# Autodesk Inventor assembly: 組合3-15
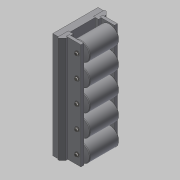
[picture p0: Inventor's stored thumbnail of the model, 180x180]
Saved by Autodesk Inventor 2018 (Build 220112000, 112)
## iProperties
Created: 2020-09-23
Part Number: 組合3-15
Material: 一般
Document SubType Name: Assembly
Designer: 王鼎鈞
Author: 王鼎鈞
## Documents named in this file (7)
- D:\2020嚴家明 功課黨\組合3-15.iam
- D:\2020嚴家明 功課黨\exercise3-11.ipt
- D:\2020嚴家明 功課黨\exercise3-12.ipt
- D:\2020嚴家明 功課黨\exercise3-13.ipt
- D:\2020嚴家明 功課黨\exercise3-14ipt.ipt
- C:\Users\王鼎鈞\Documents\Inventor\Content Center Files\R2018\zh-TW\CNS 4411\CNS 4411 - M 10 x 40.ipt
- D:\2020嚴家明 功課黨\AS 1427 - M10 x 50(4).ipt
## Components (30 placed, 6 different names)
1. exercise3-11:1 — 插入:2, 貼合:14, 插入:17, 插入:22
2. exercise3-12:1 — 貼合:9, 貼合:10, 齊平:5, 插入:1, 插入:2, 插入:3, 插入:4, 插入:5
3. exercise3-13:1 — 貼合:5, 貼合:6, 齊平:3, 貼合:9, 貼合:10, 齊平:5
4. exercise3-14ipt:1 — 貼合:5, 貼合:6, 齊平:3, 貼合:7, 貼合:8, 齊平:4, 插入:6, 插入:7, 插入:8, 插入:9, 插入:10, 插入:11, 插入:12, 插入:13, 插入:14, 插入:15
5. exercise3-13:2 — 貼合:7, 貼合:8, 齊平:4, 貼合:11, 貼合:12, 齊平:6
6. exercise3-12:2 — 貼合:11, 貼合:12, 齊平:6, 貼合:13, 貼合:14, 貼合:15, 貼合:16, 貼合:17
7. exercise3-11:2 — 插入:1, 貼合:13, 插入:16, 插入:21
8. exercise3-11:3 — 插入:3, 貼合:15, 插入:19, 插入:24
9. exercise3-11:4 — 插入:4, 貼合:16, 插入:18, 插入:23
10. exercise3-11:5 — 插入:5, 貼合:17, 插入:20, 插入:25
11. CNS 4411 M 10 x 40:1 — 插入:6
12. CNS 4411 M 10 x 40:2 — 插入:13
13. CNS 4411 M 10 x 40:3 — 插入:15
14. CNS 4411 M 10 x 40:4 — 插入:7
15. CNS 4411 M 10 x 40:5 — 插入:8
16. CNS 4411 M 10 x 40:6 — 插入:9
17. CNS 4411 M 10 x 40:7 — 插入:14
18. CNS 4411 M 10 x 40:8 — 插入:12
19. CNS 4411 M 10 x 40:9 — 插入:11
20. CNS 4411 M 10 x 40:10 — 插入:10
21. AS 1427 - M10 x 50(4):1 — 插入:18
22. AS 1427 - M10 x 50(4):2 — 插入:17
23. AS 1427 - M10 x 50(4):3 — 插入:16
24. AS 1427 - M10 x 50(4):4 — 插入:19
25. AS 1427 - M10 x 50(4):5 — 插入:20
26. AS 1427 - M10 x 50(4):6 — 插入:24
27. AS 1427 - M10 x 50(4):7 — 插入:25
28. AS 1427 - M10 x 50(4):8 — 插入:23
29. AS 1427 - M10 x 50(4):9 — 插入:22
30. AS 1427 - M10 x 50(4):10 — 插入:21
## Relationships (42: Insert 25, Mate 13, Flush 4)
- 貼合:5 [Mate]: exercise3-13:1 ↔ exercise3-14ipt:1
- 貼合:6 [Mate]: exercise3-13:1 ↔ exercise3-14ipt:1
- 齊平:3 [Flush]: exercise3-13:1 ↔ exercise3-14ipt:1
- 貼合:7 [Mate]: exercise3-14ipt:1 ↔ exercise3-13:2
- 貼合:8 [Mate]: exercise3-14ipt:1 ↔ exercise3-13:2
- 齊平:4 [Flush]: exercise3-14ipt:1 ↔ exercise3-13:2
- 貼合:9 [Mate]: exercise3-12:1 ↔ exercise3-13:1
- 貼合:10 [Mate]: exercise3-12:1 ↔ exercise3-13:1
- 齊平:5 [Flush]: exercise3-12:1 ↔ exercise3-13:1
- 貼合:11 [Mate]: exercise3-13:2 ↔ exercise3-12:2
- 貼合:12 [Mate]: exercise3-13:2 ↔ exercise3-12:2
- 齊平:6 [Flush]: exercise3-13:2 ↔ exercise3-12:2
- 插入:1 [Insert]: exercise3-12:1 ↔ exercise3-11:2
- 貼合:13 [Mate]: exercise3-12:2 ↔ exercise3-11:2
- 插入:2 [Insert]: exercise3-11:1 ↔ exercise3-12:1
- 貼合:14 [Mate]: exercise3-11:1 ↔ exercise3-12:2
- 插入:3 [Insert]: exercise3-12:1 ↔ exercise3-11:3
- 貼合:15 [Mate]: exercise3-12:2 ↔ exercise3-11:3
- 插入:4 [Insert]: exercise3-12:1 ↔ exercise3-11:4
- 貼合:16 [Mate]: exercise3-12:2 ↔ exercise3-11:4
- 插入:5 [Insert]: exercise3-12:1 ↔ exercise3-11:5
- 貼合:17 [Mate]: exercise3-12:2 ↔ exercise3-11:5
- 插入:6 [Insert]: exercise3-14ipt:1 ↔ CNS 4411 M 10 x 40:1
- 插入:7 [Insert]: exercise3-14ipt:1 ↔ CNS 4411 M 10 x 40:4
- 插入:8 [Insert]: exercise3-14ipt:1 ↔ CNS 4411 M 10 x 40:5
- 插入:9 [Insert]: exercise3-14ipt:1 ↔ CNS 4411 M 10 x 40:6
- 插入:10 [Insert]: exercise3-14ipt:1 ↔ CNS 4411 M 10 x 40:10
- 插入:11 [Insert]: exercise3-14ipt:1 ↔ CNS 4411 M 10 x 40:9
- 插入:12 [Insert]: exercise3-14ipt:1 ↔ CNS 4411 M 10 x 40:8
- 插入:13 [Insert]: exercise3-14ipt:1 ↔ CNS 4411 M 10 x 40:2
- 插入:14 [Insert]: exercise3-14ipt:1 ↔ CNS 4411 M 10 x 40:7
- 插入:15 [Insert]: exercise3-14ipt:1 ↔ CNS 4411 M 10 x 40:3
- 插入:16 [Insert]: exercise3-11:2 ↔ AS 1427 - M10 x 50(4):3
- 插入:17 [Insert]: exercise3-11:1 ↔ AS 1427 - M10 x 50(4):2
- 插入:18 [Insert]: exercise3-11:4 ↔ AS 1427 - M10 x 50(4):1
- 插入:19 [Insert]: exercise3-11:3 ↔ AS 1427 - M10 x 50(4):4
- 插入:20 [Insert]: exercise3-11:5 ↔ AS 1427 - M10 x 50(4):5
- 插入:21 [Insert]: exercise3-11:2 ↔ AS 1427 - M10 x 50(4):10
- 插入:22 [Insert]: exercise3-11:1 ↔ AS 1427 - M10 x 50(4):9
- 插入:23 [Insert]: exercise3-11:4 ↔ AS 1427 - M10 x 50(4):8
- 插入:24 [Insert]: exercise3-11:3 ↔ AS 1427 - M10 x 50(4):6
- 插入:25 [Insert]: exercise3-11:5 ↔ AS 1427 - M10 x 50(4):7
